# Autodesk Inventor assembly: EnclosurePopulated
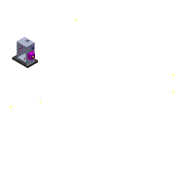
[picture p0: Inventor's stored thumbnail of the model, 180x180]
Saved by Autodesk Inventor 2017 (Build 210142000, 142)
## iProperties
Created: 2017-11-10
Part Number: EnclosurePopulated
Document SubType Name: Assembly
Designer: Kathryn Rosie
Author: Kathryn Rosie
## Documents named in this file (4)
- C:\Users\Kathryn Rosie\Google Drive\HERA\hera-cad-0\Node\Tender Model\EnclosurePopulated.iam
- C:\Users\Kathryn Rosie\Google Drive\HERA\hera-cad-0\Node\Tender Model\EnclosureAssy.iam
- C:\Users\Kathryn Rosie\Google Drive\HERA\hera-cad-0\Node\Tender Model\nodeContents.iam
- C:\Users\Kathryn Rosie\Google Drive\HERA\hera-cad-0\Node\Tender Model\plinth.ipt
## Components (3 placed, 3 different names)
1. EnclosureAssy:1 [sub-assembly] — Mate:1, Mate:2, Mate:3, Mate:4, Angle:1
2. nodeContents:1 [sub-assembly] — Mate:1, Mate:2
3. plinth:1 — Mate:3, Mate:4, Angle:1
## Relationships (5: Mate 4, Angle 1)
- Mate:1: EnclosureAssy:1 ↔ nodeContents:1
- Mate:2: EnclosureAssy:1 ↔ nodeContents:1
- Mate:3: EnclosureAssy:1 ↔ plinth:1
- Mate:4: EnclosureAssy:1 ↔ plinth:1
- Angle:1 (0 deg): EnclosureAssy:1 ↔ plinth:1
